# Autodesk Inventor assembly: Arikata
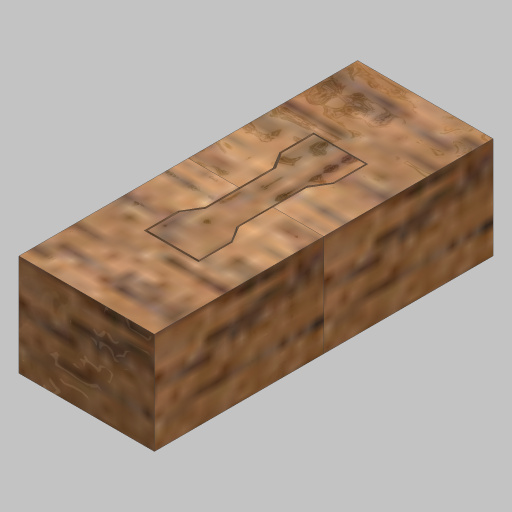
[picture p0: Inventor's stored thumbnail of the model, 512x512]
Saved by Autodesk Inventor 2023 (Build 270158000, 158)
## iProperties
Created: 2026-07-03
Part Number: Arikata
Document SubType Name: Assembly
Designer: MARTIN MAESTRE
Author: MARTIN MAESTRE
## Documents named in this file (3)
- C:\Users\MARTIN MAESTRE\OneDrive - Universidad de los Andes\POSTGRADO\202610\MAESTRIA\PROBLEMA ESPECIAL\CADS_TOLERANCIAS\Repositorio\Arikata\Arikata.iam
- C:\Users\MARTIN MAESTRE\OneDrive - Universidad de los Andes\POSTGRADO\202610\MAESTRIA\PROBLEMA ESPECIAL\CADS_TOLERANCIAS\Repositorio\Arikata\Bases.ipt
- C:\Users\MARTIN MAESTRE\OneDrive - Universidad de los Andes\POSTGRADO\202610\MAESTRIA\PROBLEMA ESPECIAL\CADS_TOLERANCIAS\Repositorio\Arikata\Spline.ipt
## Components (3 placed, 2 different names)
1. Bases:1 — Coincidencia:1, Coincidencia:2, Coincidencia:3, Nivelación:1, Nivelación:2, Coincidencia:4, Coincidencia:5
2. Bases:2 — Nivelación:1, Nivelación:2, Coincidencia:4
3. Spline:1 — Coincidencia:5
## Relationships (7: Mate 5, Flush 2)
- Coincidencia:1 [Mate]: Bases:1
- Coincidencia:2 [Mate]: Bases:1
- Coincidencia:3 [Mate]: Bases:1
- Nivelación:1 [Flush]: Bases:1 ↔ Bases:2
- Nivelación:2 [Flush]: Bases:1 ↔ Bases:2
- Coincidencia:4 [Mate]: Bases:1 ↔ Bases:2
- Coincidencia:5 [Mate]: Bases:1 ↔ Spline:1
